# Autodesk Inventor assembly: saltChute
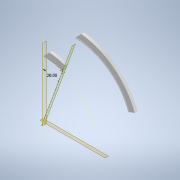
[picture p0: Inventor's stored thumbnail of the model, 180x180]
Saved by Autodesk Inventor 2021.1 (Build 251245010, 245A)
## iProperties
Created: 2020-10-17
Part Number: saltChute
Document SubType Name: Assembly
Designer: robst
Author: robst
## Documents named in this file (3)
- C:\git\CAD-Development\robSteele\HouseProjects\SaltChute\saltChute.iam
- C:\git\CAD-Development\robSteele\HouseProjects\SaltChute\SideA.ipt
- C:\git\CAD-Development\robSteele\HouseProjects\SaltChute\SideA_MIR.ipt
## Components (2 placed, 2 different names)
1. SideA:1 — Flush:1
2. SideA_MIR:1 — Mate:1
## Relationships (2: Flush 1, Mate 1)
- Flush:1 (127 mm): SideA:1
- Mate:1 (127 mm): SideA_MIR:1
